# Autodesk Inventor assembly: Switch_Micro-Lever
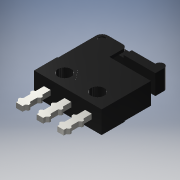
[picture p0: Inventor's stored thumbnail of the model, 180x180]
Saved by Autodesk Inventor 2018 (Build 220112000, 112)
## iProperties
Created: 2013-04-17
Part Number: Switch_Micro-Lever
Description: STEP AP203
Document SubType Name: Assembly
Designer: Bradley
Sending System: SolidWorks 2011
Preprocessor: SwSTEP 2.0
Title: D2MQ_4L_1.STEP
Revision Number: ANY
## Documents named in this file (4)
- C:\Users\Bradley\Documents\GitHub\Resources\ComponentModels\Electronics\Switch_Micro-Lever.iam
- C:\Users\Bradley\Documents\GitHub\Resources\ComponentModels\Electronics\Components\Switch_Micro-Lever\D2MQ_4L_1_BASE.ipt
- C:\Users\Bradley\Documents\GitHub\Resources\ComponentModels\Electronics\Components\Switch_Micro-Lever\D2MQ_4L_1_BUTTON.ipt
- C:\Users\Bradley\Documents\GitHub\Resources\ComponentModels\Electronics\Components\Switch_Micro-Lever\D2MQ_4L_1_ACTUATOR.ipt
## Components (3 placed, 3 different names)
1. D2MQ_4L_1_BASE_Default_1 — Insert:1, Angle:1
2. D2MQ_4L_1_BUTTON_Default_2
3. D2MQ_4L_1_ACTUATOR_Default_3 — Insert:1, Angle:1
## Relationships (2: Insert 1, Angle 1)
- Insert:1 (0.05 mm): D2MQ_4L_1_BASE_Default_1 ↔ D2MQ_4L_1_ACTUATOR_Default_3
- Angle:1 (0.1825 deg): D2MQ_4L_1_BASE_Default_1 ↔ D2MQ_4L_1_ACTUATOR_Default_3
